# Autodesk Inventor assembly: BatteryPack
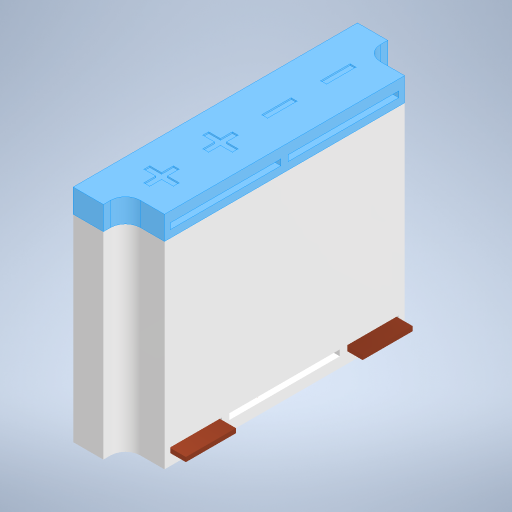
[picture p0: Inventor's stored thumbnail of the model, 512x512]
Saved by Autodesk Inventor 2023 (Build 270158000, 158)
## iProperties
Created: 2022-08-09
Part Number: BatteryPack
Document SubType Name: Assembly
Designer: Aditya Bansal
Author: Aditya Bansal
## Documents named in this file (6)
- D:\Code_Area\rocketry-datasat\structure\Electronics_Structure\Battery_V1\BatteryPack_v2.iam
- D:\Code_Area\rocketry-datasat\structure\Electronics_Structure\COTS\Battery_Cell_18650.ipt
- D:\Code_Area\rocketry-datasat\structure\Electronics_Structure\Battery_V1\Tabs\LargeTab.ipt
- D:\Code_Area\rocketry-datasat\structure\Electronics_Structure\Battery_V1\Tabs\SmallTab.ipt
- D:\Code_Area\rocketry-datasat\structure\Electronics_Structure\Battery_V1\BatteryHolderEnd_v2.ipt
- D:\Code_Area\rocketry-datasat\structure\Electronics_Structure\Battery_V1\BatteryHolderEndSeries_v2.ipt
## Components (11 placed, 5 different names)
1. Battery_Cell_18650:1 — Flush:2, Mate:47, Mate:48
2. Battery_Cell_18650:2 — Flush:1
3. Battery_Cell_18650:3 — Flush:1, Flush:3
4. Battery_Cell_18650:4 — Flush:2, Flush:3
5. BatteryHolderEnd_v2:1
6. BatteryHolderEndSeries_v2:1
7. LargeTab:1
8. LargeTab:2
9. SmallTab:2 — Mate:47
10. LargeTab:3 — Mate:48
11. SmallTab:3
## Relationships (24: Mate 21, Flush 3)
- Flush:1: Battery_Cell_18650:2 ↔ Battery_Cell_18650:3
- Flush:2: Battery_Cell_18650:1 ↔ Battery_Cell_18650:4
- Flush:3: Battery_Cell_18650:3 ↔ Battery_Cell_18650:4
- [Mate]: Battery_Cell_18650:1 ↔ BatteryHolderEndSeries_v2:1
- [Mate]: Battery_Cell_18650:2 ↔ BatteryHolderEndSeries_v2:1
- [Mate]: Battery_Cell_18650:2 ↔ BatteryHolderEnd_v2:1
- [Mate]: Battery_Cell_18650:1 ↔ BatteryHolderEnd_v2:1
- [Mate]: BatteryHolderEndSeries_v2:1 ↔ LargeTab:1
- [Mate]: BatteryHolderEndSeries_v2:1 ↔ LargeTab:1
- [Mate] (0.25 mm): BatteryHolderEndSeries_v2:1 ↔ LargeTab:1
- [Mate]: BatteryHolderEndSeries_v2:1 ↔ LargeTab:3
- [Mate]: BatteryHolderEndSeries_v2:1 ↔ LargeTab:3
- [Mate] (0.25 mm): BatteryHolderEndSeries_v2:1 ↔ LargeTab:3
- [Mate]: BatteryHolderEnd_v2:1 ↔ LargeTab:2
- [Mate] (0.25 mm): BatteryHolderEnd_v2:1 ↔ LargeTab:2
- [Mate]: BatteryHolderEnd_v2:1 ↔ LargeTab:2
- [Mate]: BatteryHolderEnd_v2:1 ↔ SmallTab:3
- [Mate]: BatteryHolderEnd_v2:1 ↔ SmallTab:3
- [Mate] (0.25 mm): BatteryHolderEnd_v2:1 ↔ SmallTab:3
- [Mate]: BatteryHolderEnd_v2:1 ↔ SmallTab:2
- [Mate]: BatteryHolderEnd_v2:1 ↔ SmallTab:2
- [Mate] (0.25 mm): BatteryHolderEnd_v2:1 ↔ SmallTab:2
- Mate:47: Battery_Cell_18650:1 ↔ SmallTab:2
- Mate:48: Battery_Cell_18650:1 ↔ LargeTab:3
